# Autodesk Inventor assembly: hypocycloid_1
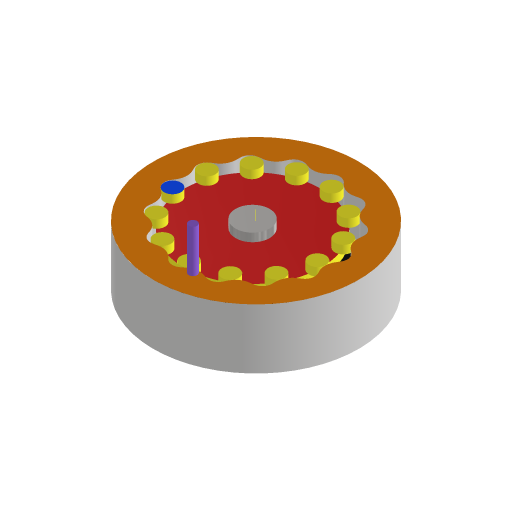
[picture p0: Inventor's stored thumbnail of the model, 512x512]
Saved by Autodesk Inventor 2023 (Build 270158000, 158)
## iProperties
Created: 2023-10-31
Part Number: hypocycloid_1
Document SubType Name: Assembly
Designer: JOU
Author: JOU
## Documents named in this file (4)
- C:\Users\JOU\Desktop\git\Special-project\Cycloidal Gear\inventor\hypocycloid_1.iam
- C:\Users\JOU\Desktop\git\Special-project\Cycloidal Gear\inventor\hypocycloid_base.ipt
- C:\Users\JOU\Desktop\git\Special-project\Cycloidal Gear\inventor\hypocycloid_InputShaft.ipt
- C:\Users\JOU\Desktop\git\Special-project\Cycloidal Gear\inventor\hypocycloid_Disk.ipt
## Components (3 placed, 3 different names)
1. hypocycloid_base:1 — 齊平:1, 齊平:2, 貼合:2
2. hypocycloid_InputShaft:1 — 貼合:1, 齊平:1, 貼合:2
3. hypocycloid_Disk:1 — 貼合:1, 齊平:2, 角度:1
## Relationships (5: Mate 2, Flush 2, Angle 1)
- 貼合:1 [Mate]: hypocycloid_InputShaft:1 ↔ hypocycloid_Disk:1
- 齊平:1 [Flush]: hypocycloid_base:1 ↔ hypocycloid_InputShaft:1
- 齊平:2 [Flush]: hypocycloid_base:1 ↔ hypocycloid_Disk:1
- 角度:1 [Angle] (772.2 deg): hypocycloid_Disk:1
- 貼合:2 [Mate]: hypocycloid_base:1 ↔ hypocycloid_InputShaft:1
